# Autodesk Inventor assembly: controler_assembly_01
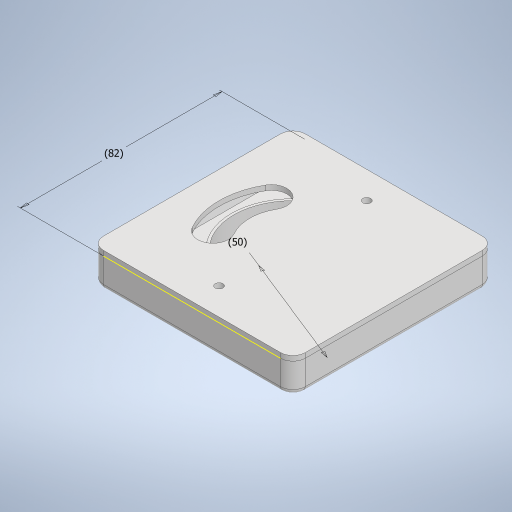
[picture p0: Inventor's stored thumbnail of the model, 512x512]
Saved by Autodesk Inventor 2023 (Build 270158000, 158)
## iProperties
Created: 2023-10-10
Part Number: controler_assembly_01
Document SubType Name: Assembly
Designer: Michal
Author: Michal
## Documents named in this file (4)
- C:\Users\Michal\Documents\Inventor\controler_assembly_01.iam
- C:\Users\Michal\Documents\Inventor\controler_01.ipt
- C:\Users\Michal\Documents\Inventor\controler_02.ipt
- C:\Users\Michal\Documents\Inventor\controler_03.ipt
## Components (3 placed, 3 different names)
1. controler_01:1 — Mate:1, Mate:2, Flush:1, Flush:2, Rigid:1, Mate:3
2. controler_02:1 — Mate:1, Rigid:1
3. controler_03:1 — Mate:2, Flush:1, Flush:2, Mate:3
## Relationships (6: Mate 3, Flush 2, WeldJoint 1)
- Mate:1: controler_01:1 ↔ controler_02:1
- Mate:2: controler_01:1 ↔ controler_03:1
- Flush:1: controler_01:1 ↔ controler_03:1
- Flush:2: controler_01:1 ↔ controler_03:1
- Rigid:1 [WeldJoint]: controler_01:1 ↔ controler_02:1
- Mate:3: controler_01:1 ↔ controler_03:1
